# Autodesk Inventor assembly: scintillatorPanel
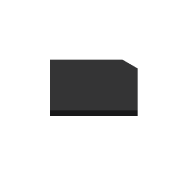
[picture p0: Inventor's stored thumbnail of the model, 180x180]
Saved by Autodesk Inventor 2017 (Build 210142000, 142)
## iProperties
Created: 2017-01-07
Part Number: scintillatorPanel
Document SubType Name: Assembly
Designer: sawaiz
Author: sawaiz
## Documents named in this file (4)
- C:\Users\sawaiz\oneDrive\projects\scintillatorPanel\scintillatorPanel.iam
- C:\Users\sawaiz\oneDrive\projects\scintillatorPanel\loopPanel.iam
- C:\Users\sawaiz\oneDrive\projects\scintillatorPanel\silvering.ipt
- C:\Users\sawaiz\oneDrive\projects\scintillatorPanel\rubberizedCoating.ipt
## Components (3 placed, 3 different names)
1. loopPanel:1 [sub-assembly] — Mate:4, Mate:5, Mate:6
2. silvering:1 — Mate:1, Mate:2, Mate:3, Mate:4, Mate:5, Mate:6
3. rubberizedCoating:1 — Mate:1, Mate:2, Mate:3
## Relationships (6: Mate 6)
- Mate:1: silvering:1 ↔ rubberizedCoating:1
- Mate:2: silvering:1 ↔ rubberizedCoating:1
- Mate:3: silvering:1 ↔ rubberizedCoating:1
- Mate:4: loopPanel:1 ↔ silvering:1
- Mate:5: loopPanel:1 ↔ silvering:1
- Mate:6: loopPanel:1 ↔ silvering:1
